# Autodesk Inventor assembly: gearbox
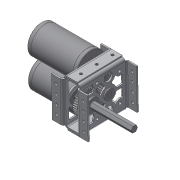
[picture p0: Inventor's stored thumbnail of the model, 180x180]
Saved by Autodesk Inventor 2013 SP1 (Build 170176100, 176)
## iProperties
Created: 2013-12-02
Part Number: gearbox
Document SubType Name: Assembly
Designer: robotics
Author: robotics
## Documents named in this file (7)
- C:\Users\robotics\Documents\GitHub\2014-Preseason-Single-Speed-Gearbox\manufacture\assemblies\gearbox.iam
- C:\Users\robotics\Documents\GitHub\2014-Preseason-Single-Speed-Gearbox\manufacture\assemblies\MotorPlate.iam
- C:\Users\robotics\Documents\GitHub\2014-Preseason-Single-Speed-Gearbox\manufacture\assemblies\NonMotorPlate.iam
- C:\Users\robotics\Documents\GitHub\2014-Preseason-Single-Speed-Gearbox\manufacture\assemblies\MiddleShaftAssembly.iam
- C:\Users\robotics\Documents\GitHub\2014-Preseason-Single-Speed-Gearbox\manufacture\assemblies\OutputShaftAssembly.iam
- C:\Users\robotics\Documents\GitHub\2014-Preseason-Single-Speed-Gearbox\manufacture\assemblies\RightMotorAssembly.iam
- C:\Users\robotics\Documents\GitHub\2014-Preseason-Single-Speed-Gearbox\manufacture\assemblies\LeftMotorAssembly.iam
## Components (6 placed, 6 different names)
1. MotorPlate:1 [sub-assembly] — Mate:12, Mate:13, Mate:14, Mate:15, Mate:16, Mate:17
2. NonMotorPlate:1 [sub-assembly]
3. MiddleShaftAssembly:1 [sub-assembly]
4. OutputShaftAssembly:1 [sub-assembly]
5. RightMotorAssembly:1 [sub-assembly] — Mate:12, Mate:13, Mate:14
6. LeftMotorAssembly:1 [sub-assembly] — Mate:15, Mate:16, Mate:17
## Relationships (14: Mate 13, Flush 1)
- [Mate]: MotorPlate:1 ↔ NonMotorPlate:1
- [Flush]: MotorPlate:1 ↔ NonMotorPlate:1
- [Mate]: MotorPlate:1 ↔ OutputShaftAssembly:1
- [Mate]: MotorPlate:1 ↔ MiddleShaftAssembly:1
- [Mate]: MotorPlate:1 ↔ MiddleShaftAssembly:1
- [Mate]: MotorPlate:1 ↔ OutputShaftAssembly:1
- [Mate]: NonMotorPlate:1 ↔ MiddleShaftAssembly:1
- [Mate]: MotorPlate:1 ↔ MiddleShaftAssembly:1
- Mate:12: MotorPlate:1 ↔ RightMotorAssembly:1
- Mate:13: MotorPlate:1 ↔ RightMotorAssembly:1
- Mate:14: MotorPlate:1 ↔ RightMotorAssembly:1
- Mate:15: MotorPlate:1 ↔ LeftMotorAssembly:1
- Mate:16: MotorPlate:1 ↔ LeftMotorAssembly:1
- Mate:17: MotorPlate:1 ↔ LeftMotorAssembly:1
